# Autodesk Inventor assembly: spool
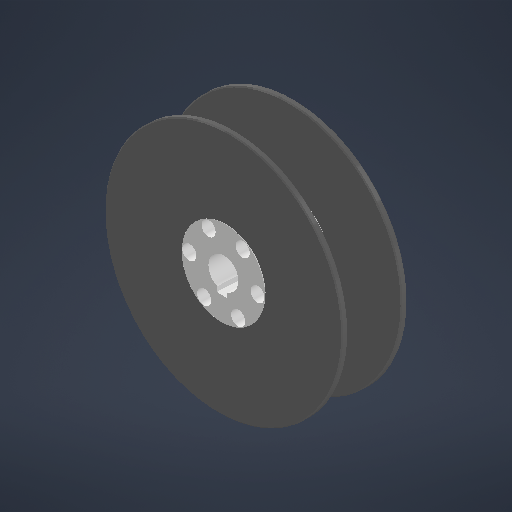
[picture p0: Inventor's stored thumbnail of the model, 512x512]
Saved by Autodesk Inventor 2026.1 (Build 301233000, 233)
## iProperties
Created: 2025-03-02
Part Number: spool
Document SubType Name: Assembly
Designer: aaron
Author: aaron
## Documents named in this file (3)
- D:\work\loopandpixel\openworkoutsystem\cad\v5\spool.iam
- D:\work\loopandpixel\openworkoutsystem\cad\v5\spool_center.ipt
- D:\work\loopandpixel\openworkoutsystem\cad\v5\spool_side.ipt
## Components (3 placed, 2 different names)
1. spool_center:1 — Insert:1, Insert:2
2. spool_side:1 — Insert:1
3. spool_side:2 — Insert:2
## Relationships (2: Insert 2)
- Insert:1: spool_center:1 ↔ spool_side:1
- Insert:2: spool_center:1 ↔ spool_side:2
